# Autodesk Inventor assembly: CREMAILLERE_2PARTIES
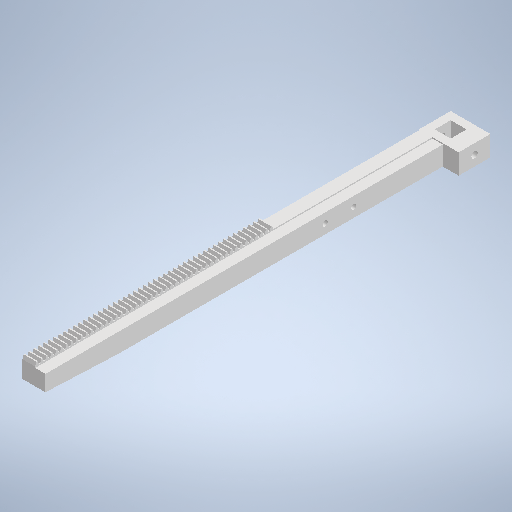
[picture p0: Inventor's stored thumbnail of the model, 512x512]
Saved by Autodesk Inventor 2025.2 (Build 292293000, 293)
## iProperties
Created: 2025-03-31
Part Number: CREMAILLERE_2PARTIES
Document SubType Name: Assembly
Designer: enezl
Author: enezl
## Documents named in this file (3)
- E:\Documents\GitHub\CDFR2025\FIPABOT\stl\CREMAILLERE_2PARTIES.iam
- E:\Documents\GitHub\CDFR2025\FIPABOT\inventor\cremaillere_partie_1.ipt
- E:\Documents\GitHub\CDFR2025\FIPABOT\inventor\cremaillere_partie_2.ipt
## Components (2 placed, 2 different names)
1. cremaillere_partie_1:1 — Glissière:1, Placage:1
2. cremaillere_partie_2:1 — Glissière:1, Placage:1
## Relationships (2: TranslationJoint 1, Mate 1)
- Glissière:1 [TranslationJoint]: cremaillere_partie_1:1 ↔ cremaillere_partie_2:1
- Placage:1 [Mate]: cremaillere_partie_1:1 ↔ cremaillere_partie_2:1
